# Autodesk Inventor assembly: Klapp-Baugruppe
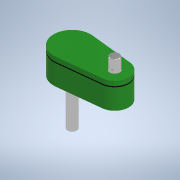
[picture p0: Inventor's stored thumbnail of the model, 180x180]
Saved by Autodesk Inventor 2021 (Build 250183000, 183)
## iProperties
Created: 2021-01-12
Part Number: Klapp-Baugruppe
Document SubType Name: Assembly
Designer: Jaro Machnow
Author: Jaro Machnow
## Documents named in this file (10)
- C:\Users\Jaro Machnow\Documents\Vault\Gruppen\Gruppe 2\Entwurf\Amphibienfahrzeug\Wechsel zwischen Land und Wasser\Wechselmechanik\Klappmechanismus\Klapp-Baugruppe.iam
- C:\Users\Jaro Machnow\Documents\Vault\Gruppen\Gruppe 2\Entwurf\Amphibienfahrzeug\Wechsel zwischen Land und Wasser\Wechselmechanik\Klappmechanismus\Klapphülle.ipt
- C:\Users\Jaro Machnow\Documents\Vault\Gruppen\Gruppe 2\Entwurf\Amphibienfahrzeug\Wechsel zwischen Land und Wasser\Wechselmechanik\Klappmechanismus\Welle1_zur_Karosserie.ipt
- C:\Users\Jaro Machnow\Documents\Vault\Gruppen\Gruppe 2\Entwurf\Amphibienfahrzeug\Wechsel zwischen Land und Wasser\Wechselmechanik\Klappmechanismus\Kraftübertragung mit Keilriemen.iam
- C:\Users\Jaro Machnow\Documents\Vault\Gruppen\Gruppe 2\Entwurf\Amphibienfahrzeug\Wechsel zwischen Land und Wasser\Wechselmechanik\Klappmechanismus\Welle2_zum_Rad.ipt
- C:\Users\Jaro Machnow\Documents\Vault\Gruppen\Gruppe 2\Entwurf\Amphibienfahrzeug\Wechsel zwischen Land und Wasser\Wechselmechanik\Klappmechanismus\Lager1.iam
- C:\Users\Jaro Machnow\Documents\Vault\Gruppen\Gruppe 2\Entwurf\Amphibienfahrzeug\Wechsel zwischen Land und Wasser\Wechselmechanik\Klappmechanismus\Keilverbindung1.iam
- C:\Users\Jaro Machnow\Documents\Vault\Gruppen\Gruppe 2\Entwurf\Amphibienfahrzeug\Wechsel zwischen Land und Wasser\Wechselmechanik\Klappmechanismus\Keilverbindung2.iam
- C:\Users\Jaro Machnow\Documents\Vault\Gruppen\Gruppe 2\Entwurf\Amphibienfahrzeug\Wechsel zwischen Land und Wasser\Wechselmechanik\Klappmechanismus\Dichtungsgummi.ipt
- C:\Users\Jaro Machnow\Documents\Vault\Gruppen\Gruppe 2\Entwurf\Amphibienfahrzeug\Wechsel zwischen Land und Wasser\Wechselmechanik\Klappmechanismus\Abdeckung.ipt
## Components (12 placed, 7 different names)
1. Welle:1 — Passend:1, Fluchtend:2, Passend:5, Fluchtend:6, Passend:10, Passend:11, Passend:12, Fluchtend:7, Winkel:1, Passend:15, Winkel:2, Passend:30
2. Kraftübertragung mit Keilriemen:1 [sub-assembly] — Passend:1, Passend:3, Passend:10, Winkel:2, Winkel:4
3. Welle:2 — Passend:3, Fluchtend:2, Passend:8, Passend:9, Passend:16, Winkel:3, Passend:17, Winkel:4, Passend:18, Passend:19, Passend:29
4. Lager:1 [sub-assembly] — Passend:5, Fluchtend:6, Passend:21
5. Lager:2 [sub-assembly] — Passend:8, Passend:9
6. Lager:3 [sub-assembly] — Passend:11, Passend:12
7. Keilverbindung:1 [sub-assembly] — Fluchtend:7, Winkel:1, Passend:15
8. Keilverbindung:2 [sub-assembly] — Passend:16, Winkel:3, Passend:17
9. Lager:4 [sub-assembly] — Passend:18, Passend:19
10. Klapphülle:1 — Passend:21, Passend:22, Passend:23, Passend:24, Passend:27, Passend:28, Passend:29, Passend:30
11. Dichtungsgummi:1 — Passend:22, Passend:23, Passend:24, Passend:25, Passend:26
12. Abdeckung:1 — Passend:25, Passend:26, Passend:27, Passend:28
## Relationships (30: Mate 23, Angle 4, Flush 3)
- Passend:1 [Mate]: Welle:1 ↔ Kraftübertragung mit Keilriemen:1
- Passend:3 [Mate]: Kraftübertragung mit Keilriemen:1 ↔ Welle:2
- Fluchtend:2 [Flush]: Welle:1 ↔ Welle:2
- Passend:5 [Mate]: Welle:1 ↔ Lager:1
- Fluchtend:6 [Flush]: Welle:1 ↔ Lager:1
- Passend:8 [Mate]: Welle:2 ↔ Lager:2
- Passend:9 [Mate]: Welle:2 ↔ Lager:2
- Passend:10 [Mate]: Welle:1 ↔ Kraftübertragung mit Keilriemen:1
- Passend:11 [Mate]: Welle:1 ↔ Lager:3
- Passend:12 [Mate]: Welle:1 ↔ Lager:3
- Fluchtend:7 [Flush] (1.0188 mm): Welle:1 ↔ Keilverbindung:1
- Winkel:1 [Angle] (0 deg): Welle:1 ↔ Keilverbindung:1
- Passend:15 [Mate]: Welle:1 ↔ Keilverbindung:1
- Winkel:2 [Angle] (174.2383 deg): Welle:1 ↔ Kraftübertragung mit Keilriemen:1
- Passend:16 [Mate] (0.9486 mm): Welle:2 ↔ Keilverbindung:2
- Winkel:3 [Angle] (0 deg): Welle:2 ↔ Keilverbindung:2
- Passend:17 [Mate]: Welle:2 ↔ Keilverbindung:2
- Winkel:4 [Angle] (146.2544 deg): Kraftübertragung mit Keilriemen:1 ↔ Welle:2
- Passend:18 [Mate]: Welle:2 ↔ Lager:4
- Passend:19 [Mate]: Welle:2 ↔ Lager:4
- Passend:21 [Mate]: Lager:1 ↔ Klapphülle:1
- Passend:22 [Mate]: Klapphülle:1 ↔ Dichtungsgummi:1
- Passend:23 [Mate]: Klapphülle:1 ↔ Dichtungsgummi:1
- Passend:24 [Mate]: Klapphülle:1 ↔ Dichtungsgummi:1
- Passend:25 [Mate]: Dichtungsgummi:1 ↔ Abdeckung:1
- Passend:26 [Mate]: Dichtungsgummi:1 ↔ Abdeckung:1
- Passend:27 [Mate]: Klapphülle:1 ↔ Abdeckung:1
- Passend:28 [Mate]: Klapphülle:1 ↔ Abdeckung:1
- Passend:29 [Mate]: Welle:2 ↔ Klapphülle:1
- Passend:30 [Mate]: Welle:1 ↔ Klapphülle:1
